# Autodesk Inventor assembly: SCSWJ10-6
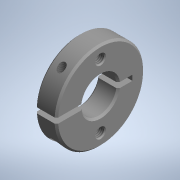
[picture p0: Inventor's stored thumbnail of the model, 180x180]
Saved by Autodesk Inventor 2022.3 (Build 263350000, 350)
## iProperties
Category: PARTsolutions
Company: MISUMI
Part Number: SCSWJ10-6
Catalog Web Link: www.cadenas.de
Description: SCSWJ, PSCSWJ, SSCSWJ-Set Collars - Slit 2 Hole/2 Tap - Compact Type - 2 Tap Type
Vendor: MISUMI
Document SubType Name: Assembly
Designer: partserver
Manufacturer: MISUMI
Mass: 2.20315 g
Surface Area: 18.7514 cm^2
Volume: 2.20315 cm^3
Density: 1 g/cm^3
PSOL_IDENT_0: {$CADENAS_DATA\23d-libs\misumi\metric\03_set_collars\scswj_asmtab.prj},193 {VTYP=3D},{STYP=ASSTAB},{
PSOL_IDENT_1: NB=SCSWJ10-6},{LINA=SCSWJ10-6},{NN=SCSWJ, PSCSWJ, SSCSWJ},{DATE=04.10.2021 04:37:38},{GEOMDATE=24.09
PSOL_IDENT_2: .2021 04:10:32},{VERSION=},{LINEID=60},{WBVAR=MAT,ST},{WBNUMERIC=}  {NB=SCSWJ10-6},{LINA=SCSWJ10-6},
PSOL_IDENT_3: {KT=DUMMY},{PN=SCSWJ10-6},{TYPE=SCSWJ},{MAT=1045},{MATA='1045','S45C Equivalent','304','SUS304 Equiv
PSOL_IDENT_4: alent'},{ST=BO},{ST0='BO','Black Oxide','ENP','Electroless Nickel Plating'},{AC=Hexagon Socket Head
PSOL_IDENT_5: Set Screw 1 Pc.},{D=10},{B=6},{D1=25},{M=M2.5},{THMD=2.5},{THDMIN=2.013},{DD=2.9},{R=2.45},{W=1.5},{
PSOL_IDENT_6: X=8.0},{Y=3},{Z=9.0},{P=18},{M1=M3},{THMD1=3},{THDMIN1=2.459},{C=0.5},{L=10},{PPATH=scswj/scswj_asmt
PSOL_IDENT_7: pl.prj}
NB: SCSWJ10-6
NN: SCSWJ, PSCSWJ, SSCSWJ
NT: Set Collars - Slit 2 Hole/2 Tap - Compact Type - 2 Tap Type
NBSYN: $PN.
LINA: SCSWJ10-6
CATALOG: Misumi
PN: SCSWJ10-6
MAT: S45C Equivalent
ST: Black Oxide
AC: Hexagon Socket Head Set Screw 1 Pc.
D: 10
B: 6
D1: 25
M: M2.5
DD: 2.9
R: 2.45
W: 1.5
X: 8
Y: 3
Z: 9
P: 18
M1: M3
SUPPLIER: MISUMI
ARTICLENO: SCSWJ10-6
BOMINFO: SCSWJ10-6
CREATOR: CADENAS GmbH
Title: SCSWJ10-6
Author: Cadenas PARTsolutions
Comments: Set Collars - Slit 2 Hole/2 Tap - Compact Type - 2 Tap Type
## Documents named in this file (3)
- C:\Users\YusukeKunita\Documents\GrabCAD\Development\BasicParts\SetCollar\SCSWJ10-6\SCSWJ10-6.iam
- C:\Users\YusukeKunita\Documents\GrabCAD\Development\BasicParts\SetCollar\SCSWJ10-6\SCSWJ10-6_b.ipt
- C:\Users\YusukeKunita\Documents\GrabCAD\Development\BasicParts\SetCollar\SCSWJ10-6\Slotted head cap screw ISO 4762 - M2_5x10.ipt
## Components (2 placed, 2 different names)
1. SCSWJ10-6_b:1 — body_screw_XY@1 <-> IP1_XY@2, body_screw_Z@1 <-> IP1_Z@2, body_screw_YZ@1 <-> IP1_YZ@2
2. Slotted head cap screw ISO 4762 - M2_5x10:1 — body_screw_XY@1 <-> IP1_XY@2, body_screw_Z@1 <-> IP1_Z@2, body_screw_YZ@1 <-> IP1_YZ@2
## Relationships (3: Mate 2, Angle 1)
- body_screw_XY@1 <-> IP1_XY@2 [Mate]: SCSWJ10-6_b:1 ↔ Slotted head cap screw ISO 4762 - M2_5x10:1
- body_screw_Z@1 <-> IP1_Z@2 [Mate]: SCSWJ10-6_b:1 ↔ Slotted head cap screw ISO 4762 - M2_5x10:1
- body_screw_YZ@1 <-> IP1_YZ@2 [Angle] (0 deg): SCSWJ10-6_b:1 ↔ Slotted head cap screw ISO 4762 - M2_5x10:1
